# Autodesk Inventor assembly: шестерни изменяемая траектория
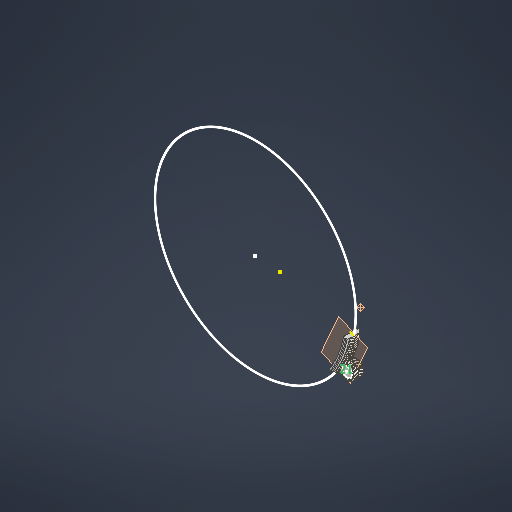
[picture p0: Inventor's stored thumbnail of the model, 512x512]
Saved by Autodesk Inventor 2026.2 (Build 302298000, 298)
## iProperties
Created: 2025-12-06
Part Number: шестерни изменяемая траектория
Document SubType Name: Assembly
Designer: Phantom
Author: Phantom
## Documents named in this file (4)
- C:\Users\Phantom\Desktop\Phantom16950\шестерни изменяемая траектория.iam
- C:\Users\Phantom\Desktop\Phantom16950\шестерни изменяемая траектория\Мастер проектирования\Цилиндрическое зубчатое зацепление2.iam
- C:\Users\Phantom\Desktop\Phantom16950\изменяемая траектория.ipt
- C:\Users\Phantom\Desktop\Phantom16950\шестерни изменяемая траектория\Мастер проектирования\Цилиндрическое зубчатое зацепление2_MIR.iam
## Components (3 placed, 3 different names)
1. Цилиндрическое зубчатое зацепление:2 [sub-assembly] — Совмещение:1, Совмещение:2, Совмещение:3, Совмещение:4, Совмещение:5
2. изменяемая траектория:1 — Совмещение:1, Совмещение:5
3. Цилиндрическое зубчатое зацепление2_MIR:1 [sub-assembly] — Совмещение:2, Совмещение:3, Совмещение:4
## Relationships (5: Mate 5)
- Совмещение:1 [Mate]: Цилиндрическое зубчатое зацепление:2 ↔ изменяемая траектория:1
- Совмещение:2 [Mate]: Цилиндрическое зубчатое зацепление:2 ↔ Цилиндрическое зубчатое зацепление2_MIR:1
- Совмещение:3 [Mate]: Цилиндрическое зубчатое зацепление:2 ↔ Цилиндрическое зубчатое зацепление2_MIR:1
- Совмещение:4 [Mate]: Цилиндрическое зубчатое зацепление:2 ↔ Цилиндрическое зубчатое зацепление2_MIR:1
- Совмещение:5 [Mate]: Цилиндрическое зубчатое зацепление:2 ↔ изменяемая траектория:1
